# Autodesk Inventor assembly: Tool Rack Assembly
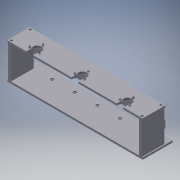
[picture p0: Inventor's stored thumbnail of the model, 180x180]
Saved by Autodesk Inventor 2019.4 (Build 234330000, 330)
## iProperties
Created: 2010-12-14
Part Number: Tool Rack Assembly
Document SubType Name: Assembly
Designer: berny
Author: berny
## Documents named in this file (7)
- C:\Users\cfang\Desktop\nebraska-silicon-lab\Hardware\General Gantry\Gantry Tool Rack\Tool Rack Assembly.iam
- C:\Users\cfang\Desktop\nebraska-silicon-lab\Hardware\General Gantry\Gantry Tool Rack\Bottom.ipt
- C:\Users\cfang\Desktop\nebraska-silicon-lab\Hardware\General Gantry\Gantry Tool Rack\Sides.ipt
- C:\Users\cfang\Desktop\nebraska-silicon-lab\Hardware\General Gantry\Gantry Tool Rack\Top.ipt
- C:\Users\cfang\Desktop\nebraska-silicon-lab\Hardware\General Gantry\Gantry Tool Rack\BackStrap1.ipt
- C:\Users\cfang\Desktop\nebraska-silicon-lab\Hardware\General Gantry\Gantry Tool Rack\84985A58.iam
- C:\Users\cfang\Desktop\nebraska-silicon-lab\Hardware\General Gantry\Gantry Tool Rack\84985A15.iam
## Components (14 placed, 6 different names)
1. Top:1 — Mate:3, Flush:13, Flush:14, Flush:15, Flush:16, Insert:33, Insert:34, Insert:35, Insert:36, Insert:37, Insert:38, Insert:39, Insert:41, Insert:42
2. Sides:1 — Mate:2, Flush:3, Flush:4, Mate:3, Flush:13, Flush:14, Mate:14
3. Sides:2 — Mate:1, Flush:15, Flush:16, Flush:17, Mate:15
4. Bottom:1 — Mate:1, Mate:2, Flush:3, Flush:4
5. BackStrap1:1 — Mate:14, Flush:17, Mate:15
6. 84985A58:1 [sub-assembly] — Insert:36
7. 84985A58:2 [sub-assembly] — Insert:38
8. 84985A58:3 [sub-assembly] — Insert:37
9. 84985A58:4 [sub-assembly] — Insert:42
10. 84985A58:5 [sub-assembly] — Insert:41
11. 84985A58:6 [sub-assembly] — Insert:39
12. 84985A15:1 [sub-assembly] — Insert:33
13. 84985A15:2 [sub-assembly] — Insert:34
14. 84985A15:3 [sub-assembly] — Insert:35
## Relationships (21: Insert 9, Flush 7, Mate 5)
- Mate:1: Sides:2 ↔ Bottom:1
- Mate:2: Sides:1 ↔ Bottom:1
- Flush:3: Sides:1 ↔ Bottom:1
- Flush:4 (3.175 mm): Sides:1 ↔ Bottom:1
- Mate:3: Top:1 ↔ Sides:1
- Flush:13 (-3.175 mm): Top:1 ↔ Sides:1
- Flush:14: Top:1 ↔ Sides:1
- Flush:15 (3.175 mm): Top:1 ↔ Sides:2
- Flush:16: Top:1 ↔ Sides:2
- Mate:14: Sides:1 ↔ BackStrap1:1
- Flush:17: Sides:2 ↔ BackStrap1:1
- Mate:15: Sides:2 ↔ BackStrap1:1
- Insert:33 (-5.08 mm): Top:1 ↔ 84985A15:1
- Insert:34 (-5.08 mm): Top:1 ↔ 84985A15:2
- Insert:35 (-5.08 mm): Top:1 ↔ 84985A15:3
- Insert:36 (-5.08 mm): Top:1 ↔ 84985A58:1
- Insert:37 (-5.08 mm): Top:1 ↔ 84985A58:3
- Insert:38 (-5.08 mm): Top:1 ↔ 84985A58:2
- Insert:39 (-5.08 mm): Top:1 ↔ 84985A58:6
- Insert:41 (-5.08 mm): Top:1 ↔ 84985A58:5
- Insert:42 (-5.08 mm): Top:1 ↔ 84985A58:4
